# Autodesk Inventor assembly: Корпус ноги в сборе_Зеркало
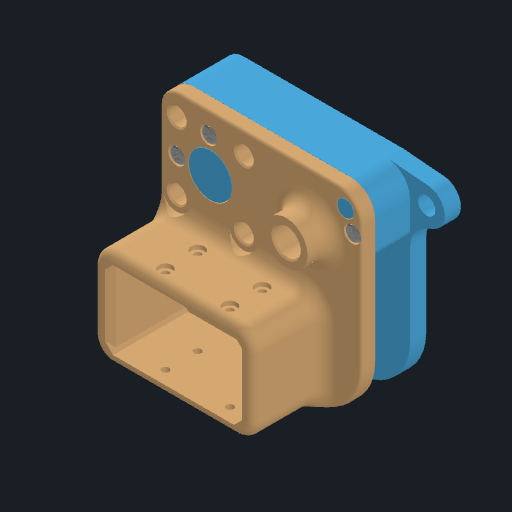
[picture p0: Inventor's stored thumbnail of the model, 512x512]
Saved by Autodesk Inventor 2025 (Build 290162010, 162A)
## iProperties
Created: 2025-01-17
Part Number: Корпус ноги в сборе_Зеркало
Document SubType Name: Assembly
Designer: Edward_Higgins
Author: Edward_Higgins
## Documents named in this file (4)
- D:\Users\Edward_Higgins\Desktop\ZAVOD\Робот Сколково\Корпус ноги в сборе_Зеркало.iam
- D:\Users\Edward_Higgins\Desktop\ZAVOD\Робот Сколково\Корпус ноги 2_Зеркало.ipt
- D:\Users\Edward_Higgins\Desktop\ZAVOD\Робот Сколково\Пластина корпуса ноги_Зеркало.ipt
- D:\Users\Edward_Higgins\Desktop\ZAVOD\Сверлильный станок\Винт М3х19.ipt
## Components (5 placed, 3 different names)
1. Корпус ноги 2_Зеркало:1 — Совмещение:2, Совмещение:1, Совмещение:5, Совмещение:4, Совмещение:3, Совмещение:7, Совмещение:6, Совмещение:12, Совмещение:11, Совмещение:10, Совмещение:9
2. Пластина корпуса ноги_Зеркало:1 — Совмещение:5, Совмещение:4, Совмещение:3
3. Винт М3х19:1 — Совмещение:7, Совмещение:6
4. Винт М3х19:2 — Совмещение:12, Совмещение:11
5. Винт М3х19:3 — Совмещение:10, Совмещение:9
## Relationships (11: Mate 11)
- Совмещение:2 [Mate]: Корпус ноги 2_Зеркало:1
- Совмещение:1 [Mate]: Корпус ноги 2_Зеркало:1
- Совмещение:5 [Mate]: Корпус ноги 2_Зеркало:1 ↔ Пластина корпуса ноги_Зеркало:1
- Совмещение:4 [Mate]: Корпус ноги 2_Зеркало:1 ↔ Пластина корпуса ноги_Зеркало:1
- Совмещение:3 [Mate]: Корпус ноги 2_Зеркало:1 ↔ Пластина корпуса ноги_Зеркало:1
- Совмещение:7 [Mate]: Корпус ноги 2_Зеркало:1 ↔ Винт М3х19:1
- Совмещение:6 [Mate]: Корпус ноги 2_Зеркало:1 ↔ Винт М3х19:1
- Совмещение:12 [Mate]: Корпус ноги 2_Зеркало:1 ↔ Винт М3х19:2
- Совмещение:11 [Mate]: Корпус ноги 2_Зеркало:1 ↔ Винт М3х19:2
- Совмещение:10 [Mate]: Корпус ноги 2_Зеркало:1 ↔ Винт М3х19:3
- Совмещение:9 [Mate]: Корпус ноги 2_Зеркало:1 ↔ Винт М3х19:3
